# Autodesk Inventor assembly: assembly
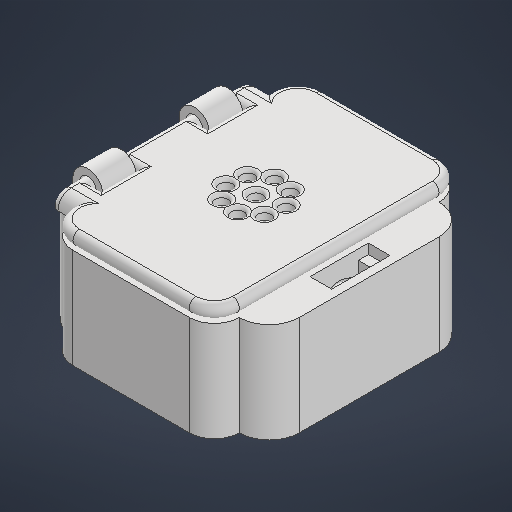
[picture p0: Inventor's stored thumbnail of the model, 512x512]
Saved by Autodesk Inventor 2026 (Build 300175050, 175E)
## iProperties
Created: 2025-05-28
Part Number: assembly
Document SubType Name: Assembly
Designer: niall
Author: niall
## Documents named in this file (4)
- C:\Users\niall\My Files\UNI_UQ\2025_SEM_1\CSSE4011\Final Project\repo\wiki_assets\files\inventor\assembly.iam
- C:\Users\niall\My Files\UNI_UQ\2025_SEM_1\CSSE4011\Final Project\repo\wiki_assets\files\inventor\box.ipt
- C:\Users\niall\My Files\UNI_UQ\2025_SEM_1\CSSE4011\Final Project\repo\wiki_assets\files\inventor\lid.ipt
- C:\Users\niall\My Files\UNI_UQ\2025_SEM_1\CSSE4011\Final Project\repo\wiki_assets\files\inventor\lid2.ipt
## Components (3 placed, 3 different names)
1. box:1 — Flush:1, Flush:2
2. lid2:1 — Flush:1
3. lid:1 — Flush:3
## Relationships (3: Flush 3)
- Flush:1: box:1 ↔ lid2:1
- Flush:2 (1 mm): box:1
- Flush:3: lid:1
